# Autodesk Inventor assembly: Hopper
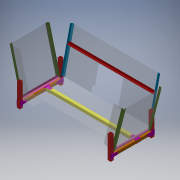
[picture p0: Inventor's stored thumbnail of the model, 180x180]
Saved by Autodesk Inventor 2017 (Build 210142000, 142)
## iProperties
Created: 2017-01-16
Part Number: Hopper
Document SubType Name: Assembly
Designer: Ben
Mass: 2513.85 g
Surface Area: 24217.2 cm^2
Volume: 1899.11 cm^3
Density: 1.3237 g/cm^3
Author: Ben
## Documents named in this file (14)
- C:\Users\Ben\Desktop\Projects\2017 Robot\Hopper\Hopper.iam
- C:\Users\Ben\Desktop\Projects\2017 Robot\Hopper\Short Side.ipt
- C:\Users\Ben\Desktop\Projects\2017 Robot\Hopper\Long Side.ipt
- C:\Users\Ben\Desktop\Projects\2017 Robot\Hopper\Upright.ipt
- C:\Users\Ben\Desktop\Projects\2017 Robot\Hopper\Short Wall support.ipt
- C:\Users\Ben\Desktop\Projects\2017 Robot\Hopper\Long Wall Support.ipt
- C:\Users\Ben\Desktop\Projects\2017 Robot\Hopper\Short Wall.ipt
- C:\Users\Ben\Desktop\Projects\2017 Robot\Hopper\Long Wall.ipt
- C:\Users\Ben\Desktop\Projects\2017 Robot\Hopper\Bottom.ipt
- C:\Users\Ben\Desktop\Projects\2017 Robot\Hopper\Bottom Sides.ipt
- C:\Users\Ben\Desktop\Projects\2017 Robot\Hopper\Side Walls.ipt
- C:\Users\Ben\Desktop\Projects\2017 Robot\Hopper\L Plate.ipt
- C:\Users\Ben\Desktop\Projects\2017 Robot\Hopper\Short Wall Cross.ipt
- C:\Users\Ben\Desktop\Projects\2017 Robot\Hopper\Long Wall Cross.ipt
## Components (36 placed, 13 different names)
1. Short Side:1 — Flush:8, Mate:5, Flush:9, Flush:15, Mate:10, Flush:17, Mate:25, Mate:26, Mate:28, Insert:8, Insert:10, Insert:12, Mate:33, Flush:32, Mate:38, Insert:31, Insert:32, Insert:34
2. Short Side:2 — Mate:4, Flush:7, Flush:8, Mate:6, Flush:11, Mate:21, Mate:23, Mate:24, Insert:18, Insert:20, Insert:22, Mate:34, Flush:33, Mate:36, Insert:29, Insert:36, Insert:38
3. Long Side:1 — Mate:33, Mate:34, Flush:32, Flush:33, Flush:34, Mate:35, Flush:35, Insert:33, Insert:35, Insert:37, Insert:39
4. Upright:1 — Flush:14, Flush:15, Mate:10, Flush:17, Insert:1, Flush:19, Flush:20, Flush:21, Insert:5, Mate:41, Mate:42, Insert:24, Insert:30
5. Upright:2 — Mate:4, Flush:7, Insert:3, Flush:21, Insert:6, Flush:34, Mate:43, Insert:27, Insert:28
6. Upright:3 — Mate:5, Flush:9, Mate:7, Flush:14, Insert:2, Flush:20, Insert:23
7. Upright:4 — Mate:6, Flush:11, Insert:4, Flush:19, Insert:25, Insert:26
8. Short Wall support:1 — Insert:1, Flush:22, Mate:13, Mate:42
9. Short Wall support:2 — Insert:2, Flush:22, Mate:14, Flush:26, Mate:31, Mate:32, Mate:48, Flush:36
10. Short Wall support:3 — Insert:3, Flush:23, Mate:12, Mate:43
11. Short Wall support:4 — Insert:4, Flush:23, Mate:11, Flush:25, Mate:44, Mate:45, Mate:46
12. Long Wall Support:1 — Insert:5, Flush:24, Flush:27, Mate:40, Mate:41
13. Long Wall Support:2 — Insert:6, Flush:24, Mate:39
14. Short Wall:1 — Mate:11, Mate:12, Flush:25, Mate:53, Flush:39, Flush:40
15. Short Wall:2 — Mate:13, Mate:14, Flush:26, Mate:50, Mate:52
16. Long Wall:1 — Flush:27, Mate:39, Mate:40, Mate:51, Flush:37, Flush:38
17. Bottom:1 — Mate:22, Mate:27, Mate:35, Mate:36, Mate:38
18. Bottom Sides:1 — Mate:21, Mate:22, Mate:23, Mate:24, Mate:47
19. Bottom Sides:2 — Mate:25, Mate:26, Mate:27, Mate:28
20. Side Walls:1 — Mate:44, Mate:45, Mate:46, Mate:47
21. Side Walls:2 — Mate:31, Mate:32, Mate:48
22. L Plate:1 — Insert:12
23. L Plate:2 — Insert:8, Insert:23
24. L Plate:3 — Insert:10, Insert:24
25. L Plate:5 — Insert:18, Insert:27
26. L Plate:7 — Insert:20, Insert:26
27. L Plate:8 — Insert:22, Insert:25
28. L Plate:9 — Insert:28, Insert:29
29. L Plate:10 — Insert:30, Insert:31
30. L Plate:11 — Insert:34, Insert:35
31. L Plate:12 — Insert:32, Insert:33
32. L Plate:13 — Insert:36, Insert:37
33. L Plate:14 — Insert:38, Insert:39
34. Short Wall Cross:1 — Mate:50, Flush:36, Mate:52
35. Long Wall Cross:1 — Mate:51, Flush:37, Flush:38
36. Short Wall Cross:2 — Mate:53, Flush:39, Flush:40
## Relationships (94: Mate 38, Insert 29, Flush 27)
- Mate:4: Short Side:2 ↔ Upright:2
- Flush:7: Short Side:2 ↔ Upright:2
- Flush:8: Short Side:1 ↔ Short Side:2
- Mate:5: Short Side:1 ↔ Upright:3
- Flush:9: Short Side:1 ↔ Upright:3
- Mate:6: Short Side:2 ↔ Upright:4
- Flush:11: Short Side:2 ↔ Upright:4
- Mate:7: Upright:3
- Flush:14: Upright:1 ↔ Upright:3
- Flush:15: Short Side:1 ↔ Upright:1
- Mate:10: Short Side:1 ↔ Upright:1
- Flush:17 (25.4 mm): Short Side:1 ↔ Upright:1
- Insert:1: Upright:1 ↔ Short Wall support:1
- Insert:2: Upright:3 ↔ Short Wall support:2
- Insert:3: Upright:2 ↔ Short Wall support:3
- Insert:4: Upright:4 ↔ Short Wall support:4
- Flush:19: Upright:1 ↔ Upright:4
- Flush:20: Upright:1 ↔ Upright:3
- Flush:21: Upright:1 ↔ Upright:2
- Flush:22: Short Wall support:1 ↔ Short Wall support:2
- Flush:23: Short Wall support:3 ↔ Short Wall support:4
- Insert:5: Upright:1 ↔ Long Wall Support:1
- Insert:6: Upright:2 ↔ Long Wall Support:2
- Flush:24: Long Wall Support:1 ↔ Long Wall Support:2
- Mate:11: Short Wall support:4 ↔ Short Wall:1
- Mate:12: Short Wall support:3 ↔ Short Wall:1
- Flush:25: Short Wall support:4 ↔ Short Wall:1
- Mate:13: Short Wall support:1 ↔ Short Wall:2
- Mate:14: Short Wall support:2 ↔ Short Wall:2
- Flush:26: Short Wall support:2 ↔ Short Wall:2
- Flush:27: Long Wall Support:1 ↔ Long Wall:1
- Flush:28 (-82.55 mm)
- Flush:29 (495.3 mm)
- Mate:21: Short Side:2 ↔ Bottom Sides:1
- Mate:22: Bottom:1 ↔ Bottom Sides:1
- Mate:23 (-6.35 mm): Short Side:2 ↔ Bottom Sides:1
- Mate:24 (85.725 mm): Short Side:2 ↔ Bottom Sides:1
- Mate:25: Short Side:1 ↔ Bottom Sides:2
- Mate:26 (-6.35 mm): Short Side:1 ↔ Bottom Sides:2
- Mate:27: Bottom:1 ↔ Bottom Sides:2
- Mate:28 (85.725 mm): Short Side:1 ↔ Bottom Sides:2
- Mate:31: Short Wall support:2 ↔ Side Walls:2
- Mate:32: Short Wall support:2 ↔ Side Walls:2
- Insert:8: Short Side:1 ↔ L Plate:2
- Insert:10: Short Side:1 ↔ L Plate:3
- Insert:12: Short Side:1 ↔ L Plate:1
- Insert:18: Short Side:2 ↔ L Plate:5
- Insert:20: Short Side:2 ↔ L Plate:7
- Insert:22: Short Side:2 ↔ L Plate:8
- Mate:33: Short Side:1 ↔ Long Side:1
- Mate:34: Short Side:2 ↔ Long Side:1
- Flush:32: Short Side:1 ↔ Long Side:1
- Flush:33: Short Side:2 ↔ Long Side:1
- Flush:34 (127 mm): Long Side:1 ↔ Upright:2
- Mate:35: Long Side:1 ↔ Bottom:1
- Mate:36 (-19.05 mm): Short Side:2 ↔ Bottom:1
- Mate:38: Short Side:1 ↔ Bottom:1
- Flush:35: Long Side:1
- Mate:39: Long Wall Support:2 ↔ Long Wall:1
- Mate:40: Long Wall Support:1 ↔ Long Wall:1
- Mate:41 (76.2 mm): Upright:1 ↔ Long Wall Support:1
- Mate:42 (88.9 mm): Upright:1 ↔ Short Wall support:1
- Mate:43 (88.9 mm): Upright:2 ↔ Short Wall support:3
- Insert:23: Upright:3 ↔ L Plate:2
- Insert:24: Upright:1 ↔ L Plate:3
- Insert:25: Upright:4 ↔ L Plate:8
- Insert:26: Upright:4 ↔ L Plate:7
- Insert:27: Upright:2 ↔ L Plate:5
- Insert:28: Upright:2 ↔ L Plate:9
- Insert:29: Short Side:2 ↔ L Plate:9
- Insert:30: Upright:1 ↔ L Plate:10
- Insert:31: Short Side:1 ↔ L Plate:10
- Insert:32: Short Side:1 ↔ L Plate:12
- Insert:33: Long Side:1 ↔ L Plate:12
- Insert:34: Short Side:1 ↔ L Plate:11
- Insert:35: Long Side:1 ↔ L Plate:11
- Insert:36: Short Side:2 ↔ L Plate:13
- Insert:37: Long Side:1 ↔ L Plate:13
- Insert:38: Short Side:2 ↔ L Plate:14
- Insert:39: Long Side:1 ↔ L Plate:14
- Mate:44: Short Wall support:4 ↔ Side Walls:1
- Mate:45: Short Wall support:4 ↔ Side Walls:1
- Mate:46: Short Wall support:4 ↔ Side Walls:1
- Mate:47 (1.5875 mm): Bottom Sides:1 ↔ Side Walls:1
- Mate:48: Short Wall support:2 ↔ Side Walls:2
- Mate:50: Short Wall:2 ↔ Short Wall Cross:1
- Flush:36 (3.175 mm): Short Wall support:2 ↔ Short Wall Cross:1
- Mate:51: Long Wall:1 ↔ Long Wall Cross:1
- Flush:37: Long Wall:1 ↔ Long Wall Cross:1
- Flush:38: Long Wall:1 ↔ Long Wall Cross:1
- Mate:52: Short Wall:2 ↔ Short Wall Cross:1
- Mate:53: Short Wall:1 ↔ Short Wall Cross:2
- Flush:39: Short Wall:1 ↔ Short Wall Cross:2
- Flush:40: Short Wall:1 ↔ Short Wall Cross:2
